# Autodesk Inventor assembly: center wheel assembly
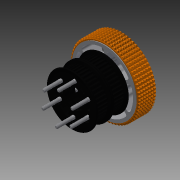
[picture p0: Inventor's stored thumbnail of the model, 180x180]
Saved by Autodesk Inventor 2014 SP1 (Build 180222100, 222)
## iProperties
Created: 2014-01-05
Part Number: center wheel assembly
Document SubType Name: Assembly
Designer: Arpan
Author: Arpan
## Documents named in this file (5)
- C:\Users\Arpan\Documents\GitHub\2014buildCAD\chassisdrivetrain\chassis light\COTS items\center wheel assembly.iam
- C:\Users\Arpan\Documents\GitHub\2014buildCAD\chassisdrivetrain\chassis light\COTS items\4 Inch Performance Wheel Tread.ipt
- C:\Users\Arpan\Documents\GitHub\2014buildCAD\chassisdrivetrain\chassis light\COTS items\4 Perf ThruTread 500 Hex (1).ipt
- C:\Users\Arpan\Documents\GitHub\2014buildCAD\chassisdrivetrain\chassis light\COTS items\DBK_42ToothPulley V2.iam
- C:\Users\Arpan\Documents\GitHub\2014buildCAD\chassisdrivetrain\chassis light\COTS items\91251A085.ipt
## Components (10 placed, 4 different names)
1. 4 Inch Performance Wheel Tread:1 — Mate:1, Mate:2
2. 4 Perf ThruTread 500 Hex (1):1 — Mate:1, Mate:2, Mate:3, Mate:4, Mate:5, Mate:6, Mate:7, Mate:8, Mate:9, Mate:10, Mate:11, Mate:12, Mate:13, Mate:14
3. DBK_42ToothPulley V2:2 [sub-assembly] — Mate:15, Mate:16, Mate:17
4. 91251A085:1 — Mate:5, Mate:14, Mate:15, Mate:19
5. 91251A085:2 — Mate:4, Mate:13
6. 91251A085:3 — Mate:3, Mate:12, Mate:16
7. 91251A085:4 — Mate:7, Mate:10, Mate:17
8. 91251A085:5 — Mate:6, Mate:11, Mate:18, Mate:20
9. 91251A085:6 — Mate:8, Mate:9
10. DBK_42ToothPulley V2:3 [sub-assembly] — Mate:18, Mate:19, Mate:20
## Relationships (20: Mate 20)
- Mate:1: 4 Inch Performance Wheel Tread:1 ↔ 4 Perf ThruTread 500 Hex (1):1
- Mate:2: 4 Inch Performance Wheel Tread:1 ↔ 4 Perf ThruTread 500 Hex (1):1
- Mate:3: 4 Perf ThruTread 500 Hex (1):1 ↔ 91251A085:3
- Mate:4: 4 Perf ThruTread 500 Hex (1):1 ↔ 91251A085:2
- Mate:5: 4 Perf ThruTread 500 Hex (1):1 ↔ 91251A085:1
- Mate:6: 4 Perf ThruTread 500 Hex (1):1 ↔ 91251A085:5
- Mate:7: 4 Perf ThruTread 500 Hex (1):1 ↔ 91251A085:4
- Mate:8: 4 Perf ThruTread 500 Hex (1):1 ↔ 91251A085:6
- Mate:9: 4 Perf ThruTread 500 Hex (1):1 ↔ 91251A085:6
- Mate:10: 4 Perf ThruTread 500 Hex (1):1 ↔ 91251A085:4
- Mate:11: 4 Perf ThruTread 500 Hex (1):1 ↔ 91251A085:5
- Mate:12: 4 Perf ThruTread 500 Hex (1):1 ↔ 91251A085:3
- Mate:13: 4 Perf ThruTread 500 Hex (1):1 ↔ 91251A085:2
- Mate:14: 4 Perf ThruTread 500 Hex (1):1 ↔ 91251A085:1
- Mate:15: DBK_42ToothPulley V2:2 ↔ 91251A085:1
- Mate:16: DBK_42ToothPulley V2:2 ↔ 91251A085:3
- Mate:17: DBK_42ToothPulley V2:2 ↔ 91251A085:4
- Mate:18: 91251A085:5 ↔ DBK_42ToothPulley V2:3
- Mate:19: 91251A085:1 ↔ DBK_42ToothPulley V2:3
- Mate:20: 91251A085:5 ↔ DBK_42ToothPulley V2:3
